# Autodesk Inventor assembly: Assembly1
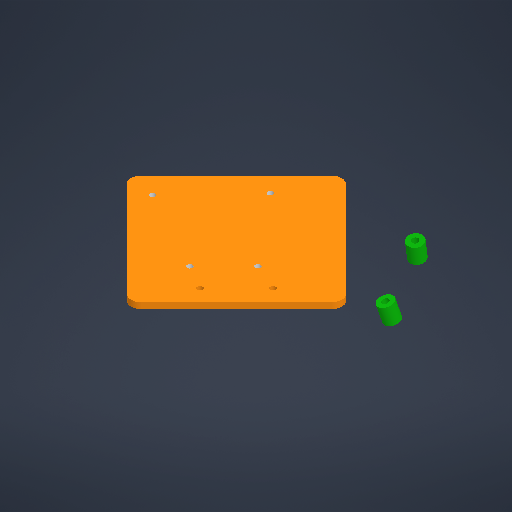
[picture p0: Inventor's stored thumbnail of the model, 512x512]
Saved by Autodesk Inventor 2026 (Build 300175000, 175)
## iProperties
Created: 2025-09-26
Part Number: Assembly1
Document SubType Name: Assembly
Designer: 7019505
Author: 7019505
## Documents named in this file (3)
- M:\Rob 30\Assembly1.iam
- H:\Scott\Robotics 30\01 Assembly Demo\main plate.ipt
- H:\Scott\Robotics 30\01 Assembly Demo\Plastic Standoff.ipt
## Components (5 placed, 2 different names)
1. main plate:2 — Mate:1, Mate:2, Mate:4, Mate:5, Mate:6
2. Plastic Standoff:1 — Mate:4
3. Plastic Standoff:2 — Mate:6
4. Plastic Standoff:3 — Mate:1, Mate:5
5. Plastic Standoff:4 — Mate:2
## Relationships (5: Mate 5)
- Mate:1: main plate:2 ↔ Plastic Standoff:3
- Mate:2: main plate:2 ↔ Plastic Standoff:4
- Mate:4: main plate:2 ↔ Plastic Standoff:1
- Mate:5: main plate:2 ↔ Plastic Standoff:3
- Mate:6: main plate:2 ↔ Plastic Standoff:2
